# Autodesk Inventor assembly: Film Applicator Valve Block
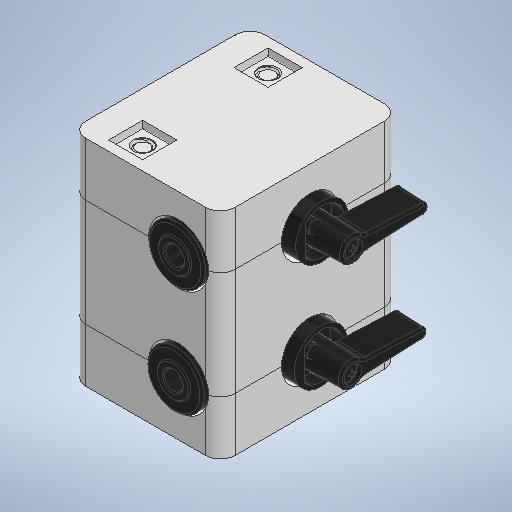
[picture p0: Inventor's stored thumbnail of the model, 512x512]
Saved by Autodesk Inventor 2025 (Build 290162000, 162)
## iProperties
Created: 2025-04-03
Part Number: Film Applicator Valve Block
Document SubType Name: Assembly
Designer: Caleb Fangmeier
Author: Caleb Fangmeier
## Documents named in this file (7)
- C:\Users\cfang\Desktop\nebraska-silicon-lab\Hardware\ETL\Jigs\Film Applicator Valve Block\Film Applicator Valve Block.iam
- C:\Users\cfang\Desktop\nebraska-silicon-lab\Hardware\ETL\Jigs\Film Applicator Valve Block\4717N12_Diverting Valve with Push-to-Connect Fittings\4717N12_Diverting Valve with Push-to-Connect Fittings.ipt
- C:\Users\cfang\Desktop\nebraska-silicon-lab\Hardware\ETL\Jigs\Film Applicator Valve Block\Valve Block Bottom.ipt
- C:\Users\cfang\Desktop\nebraska-silicon-lab\Hardware\General Gantry\Splitter Mount\90128A255_Zinc-Plated Alloy Steel Socket Head Screw\90128A255_Zinc-Plated Alloy Steel Socket Head Screw.ipt
- C:\Users\cfang\Desktop\nebraska-silicon-lab\Hardware\ETL\Jigs\Film Applicator Valve Block\Valve Block Middle.ipt
- C:\Users\cfang\Desktop\nebraska-silicon-lab\Hardware\ETL\Jigs\Film Applicator Valve Block\Valve Block Top.ipt
- C:\Users\cfang\Desktop\nebraska-silicon-lab\Hardware\General Gantry\Splitter Mount\94855A247_Low-Strength Steel Square Nut\94855A247_Low-Strength Steel Square Nut.ipt
## Components (9 placed, 6 different names)
1. 4717N12_Diverting Valve with Push-to-Connect Fittings:1 — Rotational:2, Angle:2
2. 4717N12_Diverting Valve with Push-to-Connect Fittings:2 — Rotational:1, Angle:1
3. Valve Block Bottom:1 — Rotational:1, Insert:1, Insert:2, Mate:1, Flush:1, Flush:2, Angle:1
4. 90128A255_Zinc-Plated Alloy Steel Socket Head Screw:1 — Insert:1
5. 90128A255_Zinc-Plated Alloy Steel Socket Head Screw:2 — Insert:2
6. Valve Block Middle:1 — Mate:1, Flush:1, Flush:2, Rotational:2, Mate:2, Flush:3, Flush:4, Angle:2
7. Valve Block Top:1 — Mate:2, Flush:3, Flush:4, Insert:3, Insert:4
8. 94855A247_Low-Strength Steel Square Nut:1 — Insert:4
9. 94855A247_Low-Strength Steel Square Nut:2 — Insert:3
## Relationships (14: Insert 4, Flush 4, RevoluteJoint 2, Mate 2, Angle 2)
- Rotational:1 [RevoluteJoint] (-1.5 mm): 4717N12_Diverting Valve with Push-to-Connect Fittings:2 ↔ Valve Block Bottom:1
- Insert:1: Valve Block Bottom:1 ↔ 90128A255_Zinc-Plated Alloy Steel Socket Head Screw:1
- Insert:2: Valve Block Bottom:1 ↔ 90128A255_Zinc-Plated Alloy Steel Socket Head Screw:2
- Mate:1: Valve Block Bottom:1 ↔ Valve Block Middle:1
- Flush:1: Valve Block Bottom:1 ↔ Valve Block Middle:1
- Flush:2: Valve Block Bottom:1 ↔ Valve Block Middle:1
- Rotational:2 [RevoluteJoint] (-1.5 mm): 4717N12_Diverting Valve with Push-to-Connect Fittings:1 ↔ Valve Block Middle:1
- Mate:2: Valve Block Middle:1 ↔ Valve Block Top:1
- Flush:3: Valve Block Middle:1 ↔ Valve Block Top:1
- Flush:4: Valve Block Middle:1 ↔ Valve Block Top:1
- Angle:1 (0 deg): 4717N12_Diverting Valve with Push-to-Connect Fittings:2 ↔ Valve Block Bottom:1
- Angle:2 (0 deg): 4717N12_Diverting Valve with Push-to-Connect Fittings:1 ↔ Valve Block Middle:1
- Insert:3: Valve Block Top:1 ↔ 94855A247_Low-Strength Steel Square Nut:2
- Insert:4: Valve Block Top:1 ↔ 94855A247_Low-Strength Steel Square Nut:1
